# Autodesk Inventor assembly: 6PinBlock
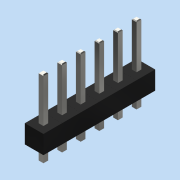
[picture p0: Inventor's stored thumbnail of the model, 180x180]
Saved by Autodesk Inventor 2017 (Build 210142000, 142)
## iProperties
Created: 2017-01-25
Part Number: 6PinBlock
Document SubType Name: Assembly
Designer: techn
Author: techn
## Documents named in this file (2)
- D:\OneDrive\Documents\Other Projects\Submarine\CAD\midships\ElectronicsSection\ServoController\6PinBlock.iam
- D:\OneDrive\Documents\Other Projects\Submarine\CAD\midships\ElectronicsSection\ServoController\3PinBlock.iam
## Components (2 placed, 1 different names)
1. 3PinBlock:1 [sub-assembly] — Mate:1, Flush:1, Flush:2
2. 3PinBlock:2 [sub-assembly] — Mate:1, Flush:1, Flush:2
## Relationships (3: Flush 2, Mate 1)
- Mate:1: 3PinBlock:1 ↔ 3PinBlock:2
- Flush:1: 3PinBlock:1 ↔ 3PinBlock:2
- Flush:2: 3PinBlock:1 ↔ 3PinBlock:2
